# Autodesk Inventor assembly: PQ60 Radio FV1.brd
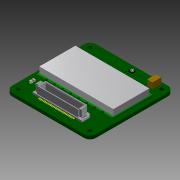
[picture p0: Inventor's stored thumbnail of the model, 180x180]
Saved by Autodesk Inventor 2015 SP1 (Build 190203100, 203)
## iProperties
Created: 2015-10-19
Part Number: PQ60 Radio FV1.brd
Document SubType Name: Assembly
Designer: Kartikye
Author: Kartikye
## Documents named in this file (8)
- C:\Users\Kartikye\Documents\GitHub\SASSat\Structure\Radio\PQ60 Radio FV1.brd.iam
- C:\Users\Kartikye\Documents\GitHub\SASSat\Structure\Radio\PQ60 Radio FV1.brd_Outline.ipt
- C:\Users\Kartikye\Documents\GitHub\SASSat\Structure\Radio\CX2156NL, CX2156NL_5.ipt
- C:\Users\Kartikye\Documents\GitHub\SASSat\Structure\Radio\MICRO-SMA, MICRO-SMA_13.ipt
- C:\Users\Kartikye\Documents\GitHub\SASSat\Structure\Radio\Radio.ipt
- C:\Users\Kartikye\Documents\GitHub\SASSat\Structure\Imported Components\0805_cap_T0.85\0805_cap_T0.85.ipt
- C:\Users\Kartikye\Documents\GitHub\SASSat\Structure\Imported Components\FX8C-60P-SV\FX8C-60P-SV.iam
- C:\Users\Kartikye\Documents\GitHub\SASSat\Structure\Imported Components\FX8C-60S-SV\FX8C-60S-SV.iam
## Components (8 placed, 8 different names)
1. PQ60 Radio FV1.brd_Outline:1 — Mate:1, Flush:1, Insert:1, Mate:2, Insert:2, Insert:3
2. C1_2
3. C2_4
4. CX2156NL_6
5. U_1_8 — Mate:1, Flush:1
6. U_4_14
7. FX8C-60P-SV:1 [sub-assembly] — Insert:1, Mate:2
8. FX8C-60S-SV:1 [sub-assembly] — Insert:2, Insert:3
## Relationships (6: Insert 3, Mate 2, Flush 1)
- Mate:1: PQ60 Radio FV1.brd_Outline:1 ↔ U_1_8
- Flush:1 (2 mm): PQ60 Radio FV1.brd_Outline:1 ↔ U_1_8
- Insert:1: PQ60 Radio FV1.brd_Outline:1 ↔ FX8C-60P-SV:1
- Mate:2: PQ60 Radio FV1.brd_Outline:1 ↔ FX8C-60P-SV:1
- Insert:2: PQ60 Radio FV1.brd_Outline:1 ↔ FX8C-60S-SV:1
- Insert:3: PQ60 Radio FV1.brd_Outline:1 ↔ FX8C-60S-SV:1
